# Autodesk Inventor assembly: battery pack
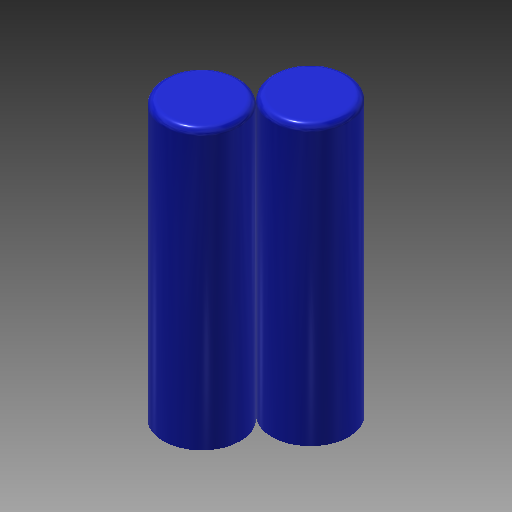
[picture p0: Inventor's stored thumbnail of the model, 512x512]
Saved by Autodesk Inventor 2017 (Build 210142000, 142)
## iProperties
Created: 2018-10-01
Part Number: battery pack
Document SubType Name: Assembly
Designer: Mitch
Author: Mitch
## Documents named in this file (2)
- E:\Youtube Channel\Pojects\Chain Blinds\Mechanical\battery pack.iam
- E:\Youtube Channel\Pojects\Chain Blinds\Mechanical\18650 Battery.ipt
## Components (2 placed, 1 different names)
1. 18650 Battery:1 — Flush:1, Tangent:1
2. 18650 Battery:2 — Flush:1, Tangent:1
## Relationships (2: Flush 1, Tangent 1)
- Flush:1: 18650 Battery:1 ↔ 18650 Battery:2
- Tangent:1: 18650 Battery:1 ↔ 18650 Battery:2
